# Autodesk Inventor assembly: FullProp
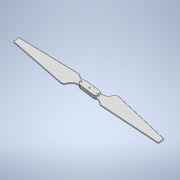
[picture p0: Inventor's stored thumbnail of the model, 180x180]
Saved by Autodesk Inventor 2022.1 (Build 261234020, 234B)
## iProperties
Created: 2022-10-16
Part Number: FullProp
Document SubType Name: Assembly
Designer: Alexander
Author: Alexander
## Documents named in this file (3)
- C:\Users\Alexander\Desktop\Drone\inventor\Propeller\FullProp.iam
- C:\Users\Alexander\Desktop\Drone\inventor\Propeller\SingleProp.ipt
- C:\Users\Alexander\Desktop\Drone\inventor\Propeller\PropConnector.ipt
## Components (4 placed, 2 different names)
1. SingleProp:1 — Rotational:1, Rotational:3
2. PropConnector:1 — Rotational:1, Rotational:2
3. SingleProp:2 — Rotational:2, Rotational:4
4. PropConnector:2 — Rotational:3, Rotational:4
## Relationships (4: RevoluteJoint 4)
- Rotational:1 [RevoluteJoint]: SingleProp:1 ↔ PropConnector:1
- Rotational:2 [RevoluteJoint]: PropConnector:1 ↔ SingleProp:2
- Rotational:3 [RevoluteJoint]: SingleProp:1 ↔ PropConnector:2
- Rotational:4 [RevoluteJoint]: SingleProp:2 ↔ PropConnector:2
